# Autodesk Inventor assembly: Full_Design
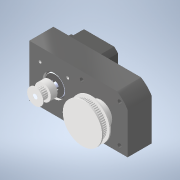
[picture p0: Inventor's stored thumbnail of the model, 180x180]
Saved by Autodesk Inventor 2022 (Build 260153000, 153)
## iProperties
Created: 2022-02-10
Part Number: Full_Design
Document SubType Name: Assembly
Designer: Mlees
Author: Mlees
## Documents named in this file (5)
- C:\Users\Mlees\Desktop\504Engineering\Stepper-Servo_Based_Robotic_Arm\Designs\Version_6\Full_Design.iam
- C:\Users\Mlees\Desktop\504Engineering\Stepper-Servo_Based_Robotic_Arm\Designs\Version_6\Downloaded_Parts\124125202-9-stp-mtr-17040w\stp-mtr-17040w.ipt
- C:\Users\Mlees\Desktop\504Engineering\Stepper-Servo_Based_Robotic_Arm\Designs\Version_6\Created_Parts\Combined_Gear_Box_modified.ipt
- C:\Users\Mlees\Desktop\504Engineering\Stepper-Servo_Based_Robotic_Arm\Designs\Version_6\Downloaded_Parts\GT2 20T Drive Pulley.ipt
- C:\Users\Mlees\Desktop\504Engineering\Stepper-Servo_Based_Robotic_Arm\Designs\Version_6\Downloaded_Parts\GT2 60T Drive Pulley.ipt
## Components (4 placed, 4 different names)
1. stp-mtr-17040w:1 — Rigid:1, Rigid:2
2. Combined_Gear_Box_modified:1 — Rigid:1, Rotational:1
3. GT2 20T Drive Pulley:1 — Rigid:2
4. GT2 60T Drive Pulley:1 — Rotational:1
## Relationships (3: WeldJoint 2, RevoluteJoint 1)
- Rigid:1 [WeldJoint]: stp-mtr-17040w:1 ↔ Combined_Gear_Box_modified:1
- Rigid:2 [WeldJoint]: stp-mtr-17040w:1 ↔ GT2 20T Drive Pulley:1
- Rotational:1 [RevoluteJoint]: Combined_Gear_Box_modified:1 ↔ GT2 60T Drive Pulley:1
